# Autodesk Inventor assembly: 新款2号螺丝+螺帽
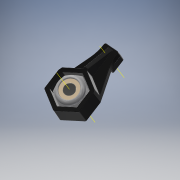
[picture p0: Inventor's stored thumbnail of the model, 180x180]
Saved by Autodesk Inventor 2019.4 (Build 234330000, 330)
## iProperties
Created: 2019-05-20
Part Number: 新款2号螺丝+螺帽
Material: 常规
Document SubType Name: Assembly
Designer: aresp
Author: aresp
## Documents named in this file (4)
- D:\2019-2020TowerTakeOverCad\ncrCadLib\新款2号螺丝+螺帽.iam
- D:\2019-2020TowerTakeOverCad\ncrCadLib\螺丝螺帽\Screw 8-32 x 0.375'' 二号.ipt
- D:\2019-2020TowerTakeOverCad\ncrCadLib\螺丝螺帽\防滑螺帽.ipt
- D:\2019-2020TowerTakeOverCad\ncrCadLib\螺丝螺帽\1-Post_Hex_Nut_Retainer_276-6482.ipt
## Components (3 placed, 3 different names)
1. 防滑螺帽:1 — 配合:2, 表面齐平:1
2. 1-Post_Hex_Nut_Retainer_276-6482:1 — 配合:1, 配合:2, 配合:3
3. Screw 8-32 x 0.375'' 二号:1 — 配合:1, 配合:3, 表面齐平:1
## Relationships (4: Mate 3, Flush 1)
- 配合:1 [Mate]: 1-Post_Hex_Nut_Retainer_276-6482:1 ↔ Screw 8-32 x 0.375'' 二号:1
- 配合:2 [Mate]: 防滑螺帽:1 ↔ 1-Post_Hex_Nut_Retainer_276-6482:1
- 配合:3 [Mate] (3.15 mm): 1-Post_Hex_Nut_Retainer_276-6482:1 ↔ Screw 8-32 x 0.375'' 二号:1
- 表面齐平:1 [Flush]: 防滑螺帽:1 ↔ Screw 8-32 x 0.375'' 二号:1
